# Autodesk Inventor assembly: 6t7000
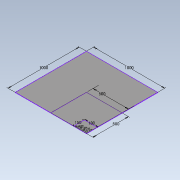
[picture p0: Inventor's stored thumbnail of the model, 180x180]
Saved by Autodesk Inventor 2020.3 (Build 243373000, 373)
## iProperties
Created: 2020-05-22
Part Number: 6t7000
Document SubType Name: Assembly
Designer: aoyama
Author: aoyama
## Documents named in this file (6)
- C:\Users\aoyam\Desktop\SRDC_local\Inventor\二年機\Geminiβ\6t7000.iam
- C:\Users\aoyam\Desktop\SRDC_local\Inventor\二年機\AL板サイズ測定板.ipt
- C:\Users\aoyam\Desktop\SRDC_local\Inventor\二年機\Geminiβ\翼\ウィング土台.ipt
- C:\Users\aoyam\Desktop\SRDC_local\Inventor\二年機\Geminiβ\腕\駆動軸.ipt
- C:\Users\aoyam\Desktop\SRDC_local\Inventor\二年機\Geminiβ\汎用部品\ｍ2歯数11ギア6td5.98.ipt
- C:\Users\aoyam\Desktop\SRDC_local\Inventor\二年機\Geminiβ\腕\アームカムAL.ipt
## Components (11 placed, 5 different names)
1. AL板サイズ測定板:1 — メイト:2, メイト:3, メイト:4, メイト:5, メイト:6, メイト:7, メイト:8, メイト:9, メイト:10, メイト:11
2. ウィング土台:1 — メイト:3, 角度:1
3. ウィング土台:2 — メイト:2, 角度:1
4. 駆動軸:1 — メイト:4
5. 駆動軸:2 — メイト:5
6. ｍ2歯数11ギア6td5.98:1 — メイト:6
7. ｍ2歯数11ギア6td5.98:2 — メイト:9
8. ｍ2歯数11ギア6td5.98:3 — メイト:7
9. ｍ2歯数11ギア6td5.98:4 — メイト:8
10. アームカムAL:1 — メイト:10
11. アームカムAL:2 — メイト:11
## Relationships (11: Mate 10, Angle 1)
- メイト:2 [Mate]: AL板サイズ測定板:1 ↔ ウィング土台:2
- メイト:3 [Mate]: AL板サイズ測定板:1 ↔ ウィング土台:1
- 角度:1 [Angle] (0 deg): ウィング土台:1 ↔ ウィング土台:2
- メイト:4 [Mate]: AL板サイズ測定板:1 ↔ 駆動軸:1
- メイト:5 [Mate]: AL板サイズ測定板:1 ↔ 駆動軸:2
- メイト:6 [Mate]: AL板サイズ測定板:1 ↔ ｍ2歯数11ギア6td5.98:1
- メイト:7 [Mate]: AL板サイズ測定板:1 ↔ ｍ2歯数11ギア6td5.98:3
- メイト:8 [Mate]: AL板サイズ測定板:1 ↔ ｍ2歯数11ギア6td5.98:4
- メイト:9 [Mate]: AL板サイズ測定板:1 ↔ ｍ2歯数11ギア6td5.98:2
- メイト:10 [Mate]: AL板サイズ測定板:1 ↔ アームカムAL:1
- メイト:11 [Mate]: AL板サイズ測定板:1 ↔ アームカムAL:2
